# Autodesk Inventor assembly: sparAssembly
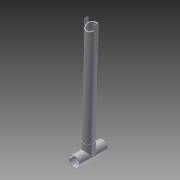
[picture p0: Inventor's stored thumbnail of the model, 180x180]
Saved by Autodesk Inventor 2014 (Build 180170000, 170)
## iProperties
Created: 2013-12-03
Part Number: sparAssembly
Document SubType Name: Assembly
Designer: Dave
Author: Dave
## Documents named in this file (4)
- C:\Users\ddeboer\Desktop\hera-cad\support\sparAssembly.iam
- C:\Users\ddeboer\Desktop\hera-cad\smallParts\pvc_T_2in.ipt
- C:\Users\ddeboer\Desktop\hera-cad\support\sparVert.ipt
- C:\Users\ddeboer\Desktop\hera-cad\smallParts\joinerBracket.ipt
## Components (4 placed, 3 different names)
1. pvc_T_2in:1 — Insert:2, Angle:1, Angle:3
2. sparVert:1 — Insert:2, Angle:1, Mate:1, Angle:2
3. joinerBracket:1 — Mate:1, Angle:2, Angle:3
4. joinerBracket:2
## Component patterns: brackets (2 elements)
## Relationships (5: Angle 3, Insert 1, Mate 1)
- Insert:2 (-25.4 mm): pvc_T_2in:1 ↔ sparVert:1
- Angle:1 (180 deg): pvc_T_2in:1 ↔ sparVert:1
- Mate:1: sparVert:1 ↔ joinerBracket:1
- Angle:2 (0 deg): sparVert:1 ↔ joinerBracket:1
- Angle:3 (0 deg): pvc_T_2in:1 ↔ joinerBracket:1
